# Autodesk Inventor assembly: Y-linear bearing shroud
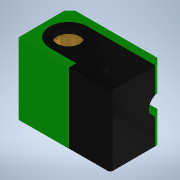
[picture p0: Inventor's stored thumbnail of the model, 180x180]
Saved by Autodesk Inventor 2020.4 (Build 244396000, 396)
## iProperties
Created: 2021-02-25
Part Number: Y-linear bearing shroud
Document SubType Name: Assembly
Designer: AOB
Mass: 36.193 g
Surface Area: 109.516 cm^2
Volume: 13.4998 cm^3
Density: 2.681 g/cm^3
Author: AOB
## Documents named in this file (4)
- C:\Users\marti\Documents\Inventor\ProjectBoron\Boron Ultima\Y-linear bearing shroud.iam
- C:\Users\marti\Documents\Inventor\ProjectBoron\Boron Ultima\lm8uu-graphite.ipt
- C:\Users\marti\Documents\Inventor\ProjectBoron\Boron Ultima\Y-linear bearing shroud-B.ipt
- C:\Users\marti\Documents\Inventor\ProjectBoron\Boron Ultima\Y-linear bearing shroud-A.ipt
## Components (3 placed, 3 different names)
1. Y-linear bearing shroud-B:1 — Cylindrical:1
2. Y-linear bearing shroud-A:3 — Cylindrical:1
3. lm8uu-graphite:1
## Relationships (4: Mate 2, Flush 1, CylindricalJoint 1)
- [Flush]: Y-linear bearing shroud-B:1 ↔ Y-linear bearing shroud-A:3
- [Mate]: Y-linear bearing shroud-A:3 ↔ lm8uu-graphite:1
- [Mate]: Y-linear bearing shroud-A:3 ↔ lm8uu-graphite:1
- Cylindrical:1: Y-linear bearing shroud-B:1 ↔ Y-linear bearing shroud-A:3
